# Autodesk Inventor assembly: Picker Tool
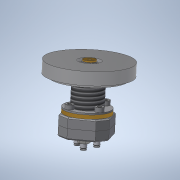
[picture p0: Inventor's stored thumbnail of the model, 180x180]
Saved by Autodesk Inventor 2022 (Build 260153000, 153)
## iProperties
Created: 2021-01-07
Part Number: Picker Tool
Document SubType Name: Assembly
Designer: caleb
Author: caleb
## Documents named in this file (7)
- C:\Users\Caleb\Desktop\nebraska-silicon-lab\Hardware\ETL\Module Assembly\Picker Tool - V2\Picker Tool - V2.iam
- C:\Users\Caleb\Desktop\nebraska-silicon-lab\Hardware\ETL\Module Assembly\Picker Tool\Picker Base.ipt
- C:\Users\Caleb\Desktop\nebraska-silicon-lab\Hardware\ETL\Module Assembly\Picker Tool\Bellows Assembly.iam
- C:\Users\Caleb\Desktop\nebraska-silicon-lab\Hardware\ETL\Module Assembly\Picker Tool\91290A119_BLACK-OXIDE CLASS 12.9 SOCKET HEAD CAP SCREW.ipt
- C:\Users\Caleb\Desktop\nebraska-silicon-lab\Hardware\ETL\Module Assembly\Picker Tool\Spool Assembly.iam
- C:\Users\Caleb\Desktop\nebraska-silicon-lab\Hardware\ETL\Module Assembly\Picker Tool\92220A311_ALLOY STEEL LOW-PROFILE SOCKET HEAD SCREW.ipt
- C:\Users\Caleb\Desktop\nebraska-silicon-lab\Hardware\ETL\Module Assembly\Picker Tool - V2\Platform Assembly - V2.iam
## Components (12 placed, 6 different names)
1. Picker Base:1 — Insert:2, Rotational:1, Cylindrical:1
2. Bellows Assembly:1 [sub-assembly] — Insert:2, Rotational:1, Insert:3, Insert:6, Insert:7, Insert:8, Insert:9, Insert:10, Insert:11, Mate:1, Mate:2
3. Platform Assembly - V2:1 [sub-assembly] — Insert:12
4. 91290A119_BLACK-OXIDE CLASS 12.9 SOCKET HEAD CAP SCREW:3 — Insert:6
5. 91290A119_BLACK-OXIDE CLASS 12.9 SOCKET HEAD CAP SCREW:4 — Insert:7
6. Spool Assembly:1 [sub-assembly] — Cylindrical:1, Insert:3, Insert:12
7. 92220A311_ALLOY STEEL LOW-PROFILE SOCKET HEAD SCREW:1 — Insert:10
8. 92220A311_ALLOY STEEL LOW-PROFILE SOCKET HEAD SCREW:2 — Insert:9
9. 92220A311_ALLOY STEEL LOW-PROFILE SOCKET HEAD SCREW:3 — Insert:11
10. 92220A311_ALLOY STEEL LOW-PROFILE SOCKET HEAD SCREW:4 — Insert:8
11. 91290A119_BLACK-OXIDE CLASS 12.9 SOCKET HEAD CAP SCREW:5 — Mate:1
12. 91290A119_BLACK-OXIDE CLASS 12.9 SOCKET HEAD CAP SCREW:6 — Mate:2
## Relationships (13: Insert 9, Mate 2, RevoluteJoint 1, CylindricalJoint 1)
- Insert:2: Picker Base:1 ↔ Bellows Assembly:1
- Rotational:1 [RevoluteJoint]: Picker Base:1 ↔ Bellows Assembly:1
- Cylindrical:1: Picker Base:1 ↔ Spool Assembly:1
- Insert:3: Bellows Assembly:1 ↔ Spool Assembly:1
- Insert:6: Bellows Assembly:1 ↔ 91290A119_BLACK-OXIDE CLASS 12.9 SOCKET HEAD CAP SCREW:3
- Insert:7: Bellows Assembly:1 ↔ 91290A119_BLACK-OXIDE CLASS 12.9 SOCKET HEAD CAP SCREW:4
- Insert:8: Bellows Assembly:1 ↔ 92220A311_ALLOY STEEL LOW-PROFILE SOCKET HEAD SCREW:4
- Insert:9: Bellows Assembly:1 ↔ 92220A311_ALLOY STEEL LOW-PROFILE SOCKET HEAD SCREW:2
- Insert:10: Bellows Assembly:1 ↔ 92220A311_ALLOY STEEL LOW-PROFILE SOCKET HEAD SCREW:1
- Insert:11: Bellows Assembly:1 ↔ 92220A311_ALLOY STEEL LOW-PROFILE SOCKET HEAD SCREW:3
- Insert:12: Platform Assembly - V2:1 ↔ Spool Assembly:1
- Mate:1: Bellows Assembly:1 ↔ 91290A119_BLACK-OXIDE CLASS 12.9 SOCKET HEAD CAP SCREW:5
- Mate:2: Bellows Assembly:1 ↔ 91290A119_BLACK-OXIDE CLASS 12.9 SOCKET HEAD CAP SCREW:6
